# Autodesk Inventor assembly: Base_Plate_Assembly
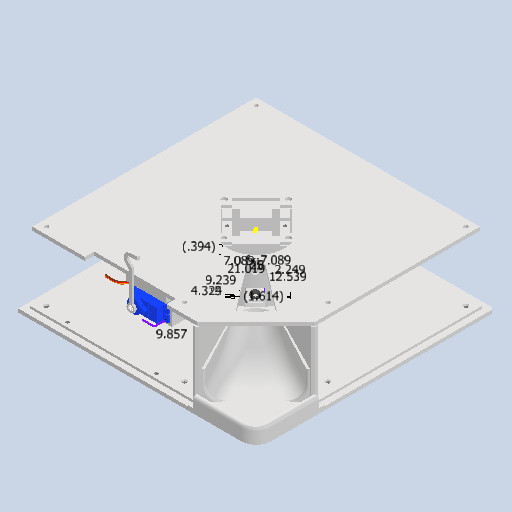
[picture p0: Inventor's stored thumbnail of the model, 512x512]
Saved by Autodesk Inventor 2022 (Build 260153000, 153)
## iProperties
Created: 2023-02-28
Part Number: Base_Plate_Assembly
Document SubType Name: Assembly
Designer: zarek
Author: zarek
## Documents named in this file (8)
- C:\Users\zarek\OneDrive\Desktop\Random New Stuff\SPB\Inside Mechanisms.iam
- C:\Users\zarek\OneDrive\Desktop\Random New Stuff\SPB\Motor_Holder.ipt
- C:\Users\zarek\OneDrive\Desktop\Random New Stuff\SPB\Drop_Plate - Copy.ipt
- C:\Users\zarek\OneDrive\Desktop\Random New Stuff\SPB\Servo&Holder.iam
- C:\Users\zarek\OneDrive\Desktop\Random New Stuff\SPB\Hook.ipt
- C:\Users\zarek\OneDrive\Desktop\Random New Stuff\SPB\Base_Plate_2_Solo_Up.ipt
- C:\Users\zarek\OneDrive\Desktop\Random New Stuff\SPB\Slide.ipt
- C:\Users\zarek\OneDrive\Desktop\Random New Stuff\SPB\Camera Assembly.iam
## Components (7 placed, 7 different names)
1. Motor_Holder:1 — Rotational:2, Rigid:3
2. Drop_Plate - Copy:1 — Rotational:2, Rotational:3
3. Servo&Holder:1 [sub-assembly] — Rotational:3, Rigid:2
4. Hook:1 — Rigid:2
5. Base_Plate_2_Solo_Up:1 — Rigid:3, Mate:2, Mate:3, Flush:1
6. Slide:1 — Mate:2
7. Camera Assembly:1 [sub-assembly] — Mate:3, Flush:1
## Relationships (7: RevoluteJoint 2, WeldJoint 2, Mate 2, Flush 1)
- Rotational:2 [RevoluteJoint]: Motor_Holder:1 ↔ Drop_Plate - Copy:1
- Rotational:3 [RevoluteJoint]: Drop_Plate - Copy:1 ↔ Servo&Holder:1
- Rigid:2 [WeldJoint]: Servo&Holder:1 ↔ Hook:1
- Rigid:3 [WeldJoint]: Motor_Holder:1 ↔ Base_Plate_2_Solo_Up:1
- Mate:2: Base_Plate_2_Solo_Up:1 ↔ Slide:1
- Mate:3: Base_Plate_2_Solo_Up:1 ↔ Camera Assembly:1
- Flush:1: Base_Plate_2_Solo_Up:1 ↔ Camera Assembly:1
